# Autodesk Inventor assembly: 36T HS Gear With Insert.ipt
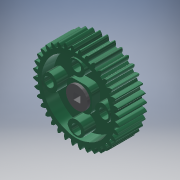
[picture p0: Inventor's stored thumbnail of the model, 180x180]
Saved by Autodesk Inventor 2019 (Build 230136000, 136)
## iProperties
Created: 2020-04-29
Part Number: 36T HS Gear With Insert.ipt
Document SubType Name: Assembly
Designer: karlv
Author: karlv
## Documents named in this file (3)
- C:\Users\karlv\Documents\VEX\62019S Repos\2020-2021_CAD\Karl CAD Lib\Gears\HS\36T HS Gear With Insert.ipt.iam
- C:\Users\karlv\Documents\VEX\62019S Repos\2020-2021_CAD\Karl CAD Lib\Gears\HS\36T HS Gear.ipt
- C:\Users\karlv\Documents\VEX\62019S Repos\2020-2021_CAD\Karl CAD Lib\Gears\Inserts\Locked Metal Inserts.ipt
## Components (3 placed, 2 different names)
1. 36T HS Gear:1 — Mate:1, Mate:2, Mate:3, Mate:4, Mate:5, Mate:6
2. Locked Metal Inserts:1 — Mate:1, Mate:2, Mate:3
3. Locked Metal Inserts:2 — Mate:4, Mate:5, Mate:6
## Relationships (6: Mate 6)
- Mate:1: 36T HS Gear:1 ↔ Locked Metal Inserts:1
- Mate:2: 36T HS Gear:1 ↔ Locked Metal Inserts:1
- Mate:3: 36T HS Gear:1 ↔ Locked Metal Inserts:1
- Mate:4: 36T HS Gear:1 ↔ Locked Metal Inserts:2
- Mate:5: 36T HS Gear:1 ↔ Locked Metal Inserts:2
- Mate:6: 36T HS Gear:1 ↔ Locked Metal Inserts:2
